# Autodesk Inventor assembly: Alignment Assembly after Cavity
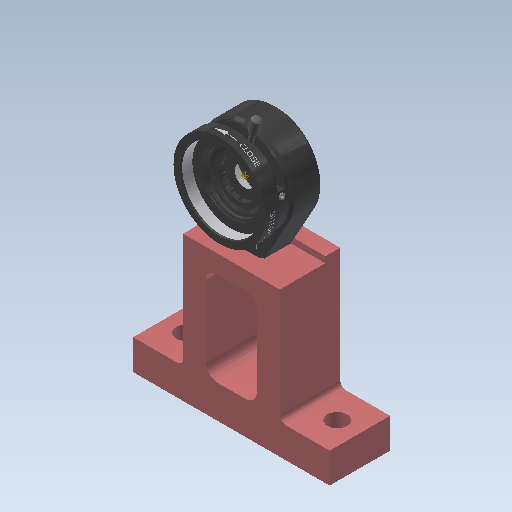
[picture p0: Inventor's stored thumbnail of the model, 512x512]
Saved by Autodesk Inventor 2020 (Build 240168000, 168)
## iProperties
Created: 2016-08-03
Part Number: Alignment Assembly after Cavity
Document SubType Name: Assembly
Designer: map
Sending System: SolidWorks 2015
Last Author: yl862
Last Saved: 2016-08-19
Author: map
## Documents named in this file (6)
- C:\Users\whgu0532\Documents\4Pi\4Pi-Oxford\Alignment Assembly after Cavity.iam
- C:\Users\whgu0532\Documents\4Pi\4Pi-Oxford\FAB-OX0002 -Lens Mount -LRM1-Vertical.ipt
- C:\Users\whgu0532\Documents\4Pi\4Pi-Oxford\Thor LMR1-M Fixed Lens Mt.ipt
- C:\Users\whgu0532\Documents\4Pi\4Pi-Oxford\SM1D12-Solidworks.ipt
- C:\Users\whgu0532\Documents\4Pi\R2017\en-US\DIN EN ISO 7092\DIN EN ISO 7092 - 5.ipt
- C:\Users\whgu0532\Documents\4Pi\4Pi-Oxford\36650.W0408.ipt
## Components (5 placed, 5 different names)
1. FAB -Len Mount -LRM1-Vertical:1 — Mate:1, Mate:2, Mate:3, Mate:9
2. Thor LMR1-M Fixed Lens Mt:1 — Mate:1, Mate:2, Mate:3, Mate:4, Mate:5
3. SM1D12-Solidworks:1 — Mate:4, Mate:5
4. 36650.W0408:1
5. DIN EN ISO 7092 5:1 — Mate:9
## Relationships (9: Mate 9)
- Mate:1: FAB -Len Mount -LRM1-Vertical:1 ↔ Thor LMR1-M Fixed Lens Mt:1
- Mate:2: FAB -Len Mount -LRM1-Vertical:1 ↔ Thor LMR1-M Fixed Lens Mt:1
- Mate:3: FAB -Len Mount -LRM1-Vertical:1 ↔ Thor LMR1-M Fixed Lens Mt:1
- Mate:4: Thor LMR1-M Fixed Lens Mt:1 ↔ SM1D12-Solidworks:1
- Mate:5: Thor LMR1-M Fixed Lens Mt:1 ↔ SM1D12-Solidworks:1
- [Mate]: 36650.W0408:1 ↔ DIN EN ISO 7092 5:1
- [Mate]: 36650.W0408:1 ↔ DIN EN ISO 7092 5:1
- [Mate]: FAB -Len Mount -LRM1-Vertical:1 ↔ 36650.W0408:1
- Mate:9: FAB -Len Mount -LRM1-Vertical:1 ↔ DIN EN ISO 7092 5:1
